# Autodesk Inventor assembly: Topside
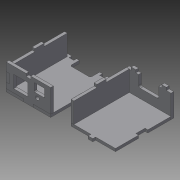
[picture p0: Inventor's stored thumbnail of the model, 180x180]
Saved by Autodesk Inventor 2015 (Build 190159000, 159)
## iProperties
Created: 2015-08-05
Part Number: Topside
Document SubType Name: Assembly
Designer: JR
Author: JR
## Documents named in this file (6)
- F:\OpenROV\2.8\Topside\Topside.iam
- F:\OpenROV\2.8\Topside\Bottom.ipt
- F:\OpenROV\2.8\Topside\RJ45Plate.ipt
- F:\OpenROV\2.8\Topside\Side.ipt
- F:\OpenROV\2.8\Topside\TerminalPlate.ipt
- F:\OpenROV\2.8\Topside\Top.ipt
## Components (6 placed, 5 different names)
1. Bottom:1 — Mate:1, Flush:1, Flush:2, Mate:2, Flush:4, Flush:8
2. RJ45Plate:1 — Flush:9, Flush:10, Flush:11
3. Side:1 — Flush:3, Mate:2, Flush:4
4. Side:2 — Flush:6, Flush:7, Mate:3, Flush:11
5. TerminalPlate:1 — Mate:1, Flush:1, Flush:2, Flush:3, Flush:5
6. Top:1 — Flush:5, Flush:6, Flush:7, Mate:3, Flush:8, Flush:9, Flush:10
## Relationships (14: Flush 11, Mate 3)
- Mate:1: Bottom:1 ↔ TerminalPlate:1
- Flush:1: Bottom:1 ↔ TerminalPlate:1
- Flush:2: Bottom:1 ↔ TerminalPlate:1
- Flush:3: Side:1 ↔ TerminalPlate:1
- Mate:2: Bottom:1 ↔ Side:1
- Flush:4: Bottom:1 ↔ Side:1
- Flush:5: TerminalPlate:1 ↔ Top:1
- Flush:6: Side:2 ↔ Top:1
- Flush:7: Side:2 ↔ Top:1
- Mate:3: Side:2 ↔ Top:1
- Flush:8: Bottom:1 ↔ Top:1
- Flush:9: RJ45Plate:1 ↔ Top:1
- Flush:10: RJ45Plate:1 ↔ Top:1
- Flush:11: RJ45Plate:1 ↔ Side:2
